# Autodesk Inventor assembly: aircilinder_15_MIR
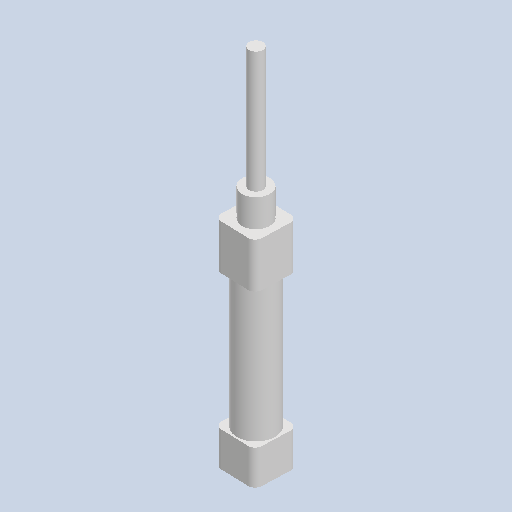
[picture p0: Inventor's stored thumbnail of the model, 512x512]
Saved by Autodesk Inventor 2024.1 (Build 281209000, 209)
## iProperties
Created: 2019-08-21
Part Number: aircilinder_15_MIR
Material: 一般
Document SubType Name: Assembly
Designer: haruy
Mass: 14.7533 g
Surface Area: 96.3525 cm^2
Volume: 10.6467 cm^3
Density: 1.38571 g/cm^3
Author: Haruka
## Documents named in this file (6)
- C:\Users\haruy\OneDrive - Kyushu University\KURT_工房共有\2023~2024\ハード\CAD\2024NHK\000_parts\エアシリンダー\airclinder\aircilinder_15_MIR.iam
- C:\Users\haruy\OneDrive - Kyushu University\KURT_工房共有\2023~2024\ハード\CAD\2024NHK\000_parts\エアシリンダー\airclinder\summer_cilinder_MIR.ipt
- C:\Users\haruy\OneDrive - Kyushu University\KURT_工房共有\2023~2024\ハード\CAD\2024NHK\000_parts\エアシリンダー\airclinder\summer_lod_MIR.ipt
- C:\Users\haruy\OneDrive - Kyushu University\KURT_工房共有\2023~2024\ハード\CAD\2024NHK\000_parts\エアシリンダー\airclinder\finger_al_mk_1_MIR.ipt
- C:\Users\haruy\OneDrive - Kyushu University\KURT_工房共有\2023~2024\ハード\CAD\2024NHK\000_parts\エアシリンダー\airclinder\finger_k_mk_1_MIR.ipt
- C:\Users\haruy\OneDrive - Kyushu University\KURT_工房共有\2023~2024\ハード\CAD\2024NHK\000_parts\エアシリンダー\airclinder\finger_k_mk_2_MIR.ipt
## Components (5 placed, 5 different names)
1. summer_cilinder_MIR:1 — 挿入:1, 角度:2, 円柱状:1
2. summer_lod_MIR:1 — 挿入:2, 円柱状:1
3. finger_al_mk_1_MIR:1 — 挿入:1, 挿入:4, 挿入:3, 角度:1
4. finger_k_mk_1_MIR:1 — 挿入:2, 角度:1
5. finger_k_mk_2_MIR:1 — 角度:2, 挿入:4, 挿入:3
## Relationships (7: Insert 4, Angle 2, CylindricalJoint 1)
- 挿入:1 [Insert]: summer_cilinder_MIR:1 ↔ finger_al_mk_1_MIR:1
- 挿入:2 [Insert] (3 mm): summer_lod_MIR:1 ↔ finger_k_mk_1_MIR:1
- 角度:2 [Angle] (0 deg): summer_cilinder_MIR:1 ↔ finger_k_mk_2_MIR:1
- 挿入:4 [Insert]: finger_al_mk_1_MIR:1 ↔ finger_k_mk_2_MIR:1
- 挿入:3 [Insert]: finger_al_mk_1_MIR:1 ↔ finger_k_mk_2_MIR:1
- 角度:1 [Angle] (0 deg): finger_al_mk_1_MIR:1 ↔ finger_k_mk_1_MIR:1
- 円柱状:1 [CylindricalJoint]: summer_cilinder_MIR:1 ↔ summer_lod_MIR:1
